# Autodesk Inventor assembly: green-house
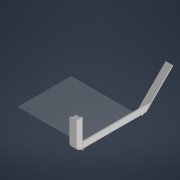
[picture p0: Inventor's stored thumbnail of the model, 180x180]
Saved by Autodesk Inventor 2021 (Build 250183000, 183)
## iProperties
Created: 2020-05-09
Part Number: green-house
Document SubType Name: Assembly
Designer: Jonathan
Author: Jonathan
## Documents named in this file (8)
- C:\Users\Jonathan\green-house\green-house.iam
- C:\Users\Jonathan\green-house\frame.ipt
- C:\Users\Jonathan\green-house\frame-roof.ipt
- C:\Users\Jonathan\green-house\frame-foot.ipt
- C:\Users\Jonathan\green-house\front-glass.ipt
- C:\Users\Jonathan\Documents\Inventor\Content Center Files\R2021\en-US\ISO 4762(2)\ISO 4762 - M3 x 12ISO.ipt
- C:\Users\Jonathan\Documents\Inventor\Content Center Files\R2021\en-US\ISO 4036(2)\ISO 4036 - M3(2).ipt
- C:\Users\Jonathan\Documents\Inventor\Content Center Files\R2021\en-US\ISO 7089\ISO 7089 - 3 - 140 HV(1).ipt
## Components (13 placed, 7 different names)
1. frame:1 — Rotational:1, Flush:1, Flush:2, Flush:3, Flush:4, Mate:1, Mate:3
2. frame-roof:1 — Rotational:1
3. frame-foot:1 — Flush:1, Flush:2
4. front-glass:1 — Flush:3, Flush:4, Mate:2
5. ISO 4762 M3 x 12:1 — Mate:1, Mate:2, Mate:4, Mate:6
6. ISO 4036 M3:1 — Mate:5, Mate:6
7. ISO 7089 3:1 — Mate:3, Mate:4, Mate:5
8. ISO 4762 M3 x 12:2
9. ISO 4036 M3:2
10. ISO 7089 3:2
11. ISO 4762 M3 x 12:3
12. ISO 4036 M3:3
13. ISO 7089 3:3
## Component patterns: (3 elements, first: ISO 4762 M3 x 12:1 + ISO 4036 M3:1 + ISO 7089 3:1)
## Relationships (11: Mate 6, Flush 4, RevoluteJoint 1)
- Rotational:1 [RevoluteJoint]: frame:1 ↔ frame-roof:1
- Flush:1: frame:1 ↔ frame-foot:1
- Flush:2: frame:1 ↔ frame-foot:1
- Flush:3: frame:1 ↔ front-glass:1
- Flush:4: frame:1 ↔ front-glass:1
- Mate:1: frame:1 ↔ ISO 4762 M3 x 12:1
- Mate:2: front-glass:1 ↔ ISO 4762 M3 x 12:1
- Mate:3: frame:1 ↔ ISO 7089 3:1
- Mate:4: ISO 4762 M3 x 12:1 ↔ ISO 7089 3:1
- Mate:5: ISO 4036 M3:1 ↔ ISO 7089 3:1
- Mate:6: ISO 4762 M3 x 12:1 ↔ ISO 4036 M3:1
